# Autodesk Inventor assembly: Default Motor Testbench Mk3
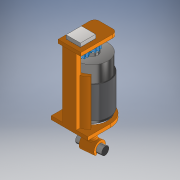
[picture p0: Inventor's stored thumbnail of the model, 180x180]
Saved by Autodesk Inventor 2018 (Build 220112000, 112)
## iProperties
Created: 2018-01-11
Part Number: Default Motor Testbench Mk3
Document SubType Name: Assembly
Designer: Moochster
Author: Moochster
## Documents named in this file (10)
- C:\Users\Moochster\OneDrive\Documents\2018 UBC\ELEC 391\Controller\CAD\Default Motor Testbench Mk3.iam
- C:\Users\Moochster\OneDrive\Documents\2018 UBC\ELEC 391\Controller\CAD\JD5B-2655W-R.ipt
- C:\Users\Moochster\OneDrive\Documents\2018 UBC\ELEC 391\Controller\CAD\Laser Mount.ipt
- C:\Users\Moochster\OneDrive\Documents\2018 UBC\ELEC 391\Controller\CAD\VLM-650-03-LPT.ipt
- C:\Users\Moochster\OneDrive\Documents\2018 UBC\ELEC 391\Controller\CAD\PEC12R-4017F-N0024.iam
- C:\Users\Moochster\OneDrive\Documents\2018 UBC\ELEC 391\Controller\CAD\Default Motor Testbench Mk3\Design Accelerator\Spur Gears1.iam
- C:\Users\Moochster\OneDrive\Documents\2018 UBC\ELEC 391\Controller\CAD\Motor Face Mount Mk2.ipt
- C:\Users\Moochster\OneDrive\Documents\2018 UBC\ELEC 391\Controller\CAD\Rotary Encoder Mount Mk2.ipt
- C:\Users\Moochster\OneDrive\Documents\2018 UBC\ELEC 391\Controller\CAD\Motor Shaft Gear.ipt
- C:\Users\Moochster\OneDrive\Documents\2018 UBC\ELEC 391\Controller\CAD\Motor Shaft Gear E.ipt
## Components (9 placed, 9 different names)
1. JD5B-2655W-R:1 — Mate:5, Mate:10, Mate:11, Angle:1, Mate:12, Mate:17, Mate:18, Mate:21, Flush:2
2. Laser Mount:1 — Mate:5, Mate:6, Mate:12, Angle:4
3. VLM-650-03-LPT:1 — Mate:6
4. PEC12R-4017F-N0024:1 [sub-assembly] — Mate:13, Mate:15, Angle:2, Mate:19, Mate:20, Mate:22, Angle:3, Mate:23
5. Motor Face Mount Mk2:1 — Mate:7, Mate:8, Mate:9, Mate:10, Mate:11, Flush:1, Mate:14, Mate:16
6. Rotary Encoder Mount Mk2:1 — Mate:13, Flush:1, Mate:14, Mate:15, Mate:16, Angle:2
7. Spur Gears:1 [sub-assembly] — Mate:17, Mate:18, Mate:19, Mate:20
8. Motor Shaft Gear E:1 — Mate:22, Angle:3, Mate:23, Rotation:1
9. Motor Shaft Gear:1 — Mate:21, Flush:2, Rotation:1, Angle:4
## Relationships (26: Mate 19, Angle 4, Flush 2, RelateRotation 1)
- Mate:5: JD5B-2655W-R:1 ↔ Laser Mount:1
- Mate:6: Laser Mount:1 ↔ VLM-650-03-LPT:1
- Mate:7: Motor Face Mount Mk2:1
- Mate:8: Motor Face Mount Mk2:1
- Mate:9: Motor Face Mount Mk2:1
- Mate:10: JD5B-2655W-R:1 ↔ Motor Face Mount Mk2:1
- Mate:11: JD5B-2655W-R:1 ↔ Motor Face Mount Mk2:1
- Angle:1 (0 deg): JD5B-2655W-R:1
- Mate:12: JD5B-2655W-R:1 ↔ Laser Mount:1
- Mate:13: PEC12R-4017F-N0024:1 ↔ Rotary Encoder Mount Mk2:1
- Flush:1: Motor Face Mount Mk2:1 ↔ Rotary Encoder Mount Mk2:1
- Mate:14: Motor Face Mount Mk2:1 ↔ Rotary Encoder Mount Mk2:1
- Mate:15: PEC12R-4017F-N0024:1 ↔ Rotary Encoder Mount Mk2:1
- Mate:16: Motor Face Mount Mk2:1 ↔ Rotary Encoder Mount Mk2:1
- Angle:2 (0 deg): PEC12R-4017F-N0024:1 ↔ Rotary Encoder Mount Mk2:1
- Mate:17: JD5B-2655W-R:1 ↔ Spur Gears:1
- Mate:18: JD5B-2655W-R:1 ↔ Spur Gears:1
- Mate:19: PEC12R-4017F-N0024:1 ↔ Spur Gears:1
- Mate:20: PEC12R-4017F-N0024:1 ↔ Spur Gears:1
- Mate:21: JD5B-2655W-R:1 ↔ Motor Shaft Gear:1
- Mate:22: PEC12R-4017F-N0024:1 ↔ Motor Shaft Gear E:1
- Angle:3 (180 deg): PEC12R-4017F-N0024:1 ↔ Motor Shaft Gear E:1
- Mate:23 (0.3 mm): PEC12R-4017F-N0024:1 ↔ Motor Shaft Gear E:1
- Flush:2 (0.5 mm): JD5B-2655W-R:1 ↔ Motor Shaft Gear:1
- Rotation:1 [RelateRotation] (1 ul): Motor Shaft Gear E:1 ↔ Motor Shaft Gear:1
- Angle:4 (0 deg): Laser Mount:1 ↔ Motor Shaft Gear:1
